# Autodesk Inventor assembly: MECANISMO DE COMPACTADO
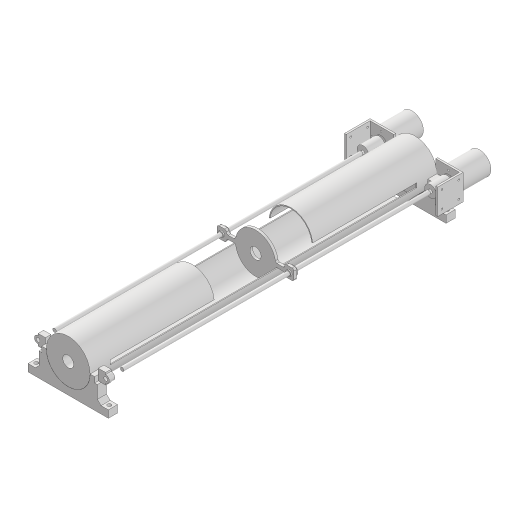
[picture p0: Inventor's stored thumbnail of the model, 512x512]
Saved by Autodesk Inventor 2024 (Build 280153000, 153)
## iProperties
Created: 2024-05-26
Part Number: MECANISMO DE COMPACTADO
Document SubType Name: Assembly
Designer: Jhuliams
Author: Jhuliams
## Documents named in this file (10)
- C:\Users\Jhuliams\Documents\GitHub\RECICLADOR_MODELO_3D\MECANISMO DE COMPACTADO\MECANISMO DE COMPACTADO.iam
- C:\Users\Jhuliams\Documents\GitHub\RECICLADOR_MODELO_3D\MECANISMO DE COMPACTADO\GUIA_DE_OBJETO.ipt
- C:\Users\Jhuliams\Documents\GitHub\RECICLADOR_MODELO_3D\MECANISMO DE COMPACTADO\TAPA QUE DESPLAZA CON TORNILLOS.ipt
- C:\Users\Jhuliams\Documents\GitHub\RECICLADOR_MODELO_3D\MECANISMO DE COMPACTADO\TUERCA DE HUSILLO.ipt
- C:\Users\Jhuliams\Documents\GitHub\RECICLADOR_MODELO_3D\MECANISMO DE COMPACTADO\TORNILLO DEPOTENCIA.ipt
- C:\Users\Jhuliams\Documents\GitHub\RECICLADOR_MODELO_3D\MECANISMO DE COMPACTADO\SOPORTE DE GUIA.ipt
- C:\Users\Jhuliams\Documents\GitHub\RECICLADOR_MODELO_3D\MECANISMO DE COMPACTADO\ACOPLE HELICOIDAL.ipt
- C:\Users\Jhuliams\Documents\GitHub\RECICLADOR_MODELO_3D\MECANISMO DE COMPACTADO\MOTOR DC.ipt
- C:\Users\Jhuliams\Documents\GitHub\RECICLADOR_MODELO_3D\MECANISMO DE COMPACTADO\SOPORTE DE MOTOR.ipt
- C:\Users\Jhuliams\Documents\GitHub\RECICLADOR_MODELO_3D\MECANISMO DE COMPACTADO\RODAMIENTO DE TORNILLO.ipt
## Components (16 placed, 9 different names)
1. GUIA_DE_OBJETO:1 — Mate:1, Mate:9, Mate:10, Mate:11, Mate:12, Mate:13, Flush:1, Flush:2
2. TAPA QUE DESPLAZA CON TORNILLOS:1 — Mate:1, Mate:3, Mate:4, Mate:5, Mate:6, Mate:11
3. TUERCA DE HUSILLO:1 — Mate:3, Mate:4, Mate:8
4. TUERCA DE HUSILLO:2 — Mate:5, Mate:6, Mate:7
5. TORNILLO DEPOTENCIA:1 — Mate:8, Mate:9, Mate:16, Mate:17, Mate:32
6. TORNILLO DEPOTENCIA:2 — Mate:7, Mate:10, Mate:14, Mate:15
7. SOPORTE DE GUIA:1 — Mate:12, Flush:1, Flush:4, Flush:5, Mate:27, Flush:6, Mate:29, Mate:30, Mate:31
8. SOPORTE DE GUIA:2 — Mate:13, Flush:2, Flush:4
9. ACOPLE HELICOIDAL:1 — Mate:14, Mate:15, Mate:19, Mate:21
10. ACOPLE HELICOIDAL:2 — Mate:16, Mate:17, Mate:18, Mate:20
11. MOTOR DC:1 — Mate:18, Mate:20, Mate:22, Mate:24
12. MOTOR DC:2 — Mate:19, Mate:21, Mate:23, Mate:25
13. SOPORTE DE MOTOR:3 — Mate:22, Mate:24, Flush:3
14. SOPORTE DE MOTOR:5 — Mate:23, Mate:25, Flush:3
15. RODAMIENTO DE TORNILLO:1 — Flush:5, Mate:27, Mate:30, Mate:32
16. RODAMIENTO DE TORNILLO:2 — Flush:6, Mate:29, Mate:31
## Relationships (35: Mate 29, Flush 6)
- Mate:1: GUIA_DE_OBJETO:1 ↔ TAPA QUE DESPLAZA CON TORNILLOS:1
- Mate:3: TAPA QUE DESPLAZA CON TORNILLOS:1 ↔ TUERCA DE HUSILLO:1
- Mate:4: TAPA QUE DESPLAZA CON TORNILLOS:1 ↔ TUERCA DE HUSILLO:1
- Mate:5: TAPA QUE DESPLAZA CON TORNILLOS:1 ↔ TUERCA DE HUSILLO:2
- Mate:6: TAPA QUE DESPLAZA CON TORNILLOS:1 ↔ TUERCA DE HUSILLO:2
- Mate:7: TUERCA DE HUSILLO:2 ↔ TORNILLO DEPOTENCIA:2
- Mate:8: TUERCA DE HUSILLO:1 ↔ TORNILLO DEPOTENCIA:1
- Mate:9: GUIA_DE_OBJETO:1 ↔ TORNILLO DEPOTENCIA:1
- Mate:10: GUIA_DE_OBJETO:1 ↔ TORNILLO DEPOTENCIA:2
- Mate:11 (1 mm): GUIA_DE_OBJETO:1 ↔ TAPA QUE DESPLAZA CON TORNILLOS:1
- Mate:12: GUIA_DE_OBJETO:1 ↔ SOPORTE DE GUIA:1
- Mate:13: GUIA_DE_OBJETO:1 ↔ SOPORTE DE GUIA:2
- Flush:1: GUIA_DE_OBJETO:1 ↔ SOPORTE DE GUIA:1
- Flush:2: GUIA_DE_OBJETO:1 ↔ SOPORTE DE GUIA:2
- Mate:14: TORNILLO DEPOTENCIA:2 ↔ ACOPLE HELICOIDAL:1
- Mate:15 (5 mm): TORNILLO DEPOTENCIA:2 ↔ ACOPLE HELICOIDAL:1
- Mate:16: TORNILLO DEPOTENCIA:1 ↔ ACOPLE HELICOIDAL:2
- Mate:17 (5 mm): TORNILLO DEPOTENCIA:1 ↔ ACOPLE HELICOIDAL:2
- Mate:18: ACOPLE HELICOIDAL:2 ↔ MOTOR DC:1
- Mate:19: ACOPLE HELICOIDAL:1 ↔ MOTOR DC:2
- Mate:20 (10 mm): ACOPLE HELICOIDAL:2 ↔ MOTOR DC:1
- Mate:21 (10 mm): ACOPLE HELICOIDAL:1 ↔ MOTOR DC:2
- Mate:22: MOTOR DC:1 ↔ SOPORTE DE MOTOR:3
- Mate:23: MOTOR DC:2 ↔ SOPORTE DE MOTOR:5
- Mate:24: MOTOR DC:1 ↔ SOPORTE DE MOTOR:3
- Mate:25: MOTOR DC:2 ↔ SOPORTE DE MOTOR:5
- Flush:3: SOPORTE DE MOTOR:3 ↔ SOPORTE DE MOTOR:5
- Flush:4: SOPORTE DE GUIA:1 ↔ SOPORTE DE GUIA:2
- Flush:5 (10 mm): SOPORTE DE GUIA:1 ↔ RODAMIENTO DE TORNILLO:1
- Mate:27: SOPORTE DE GUIA:1 ↔ RODAMIENTO DE TORNILLO:1
- Flush:6 (10 mm): SOPORTE DE GUIA:1 ↔ RODAMIENTO DE TORNILLO:2
- Mate:29: SOPORTE DE GUIA:1 ↔ RODAMIENTO DE TORNILLO:2
- Mate:30: SOPORTE DE GUIA:1 ↔ RODAMIENTO DE TORNILLO:1
- Mate:31: SOPORTE DE GUIA:1 ↔ RODAMIENTO DE TORNILLO:2
- Mate:32: TORNILLO DEPOTENCIA:1 ↔ RODAMIENTO DE TORNILLO:1
